# Autodesk Inventor assembly: suspensionsystem1
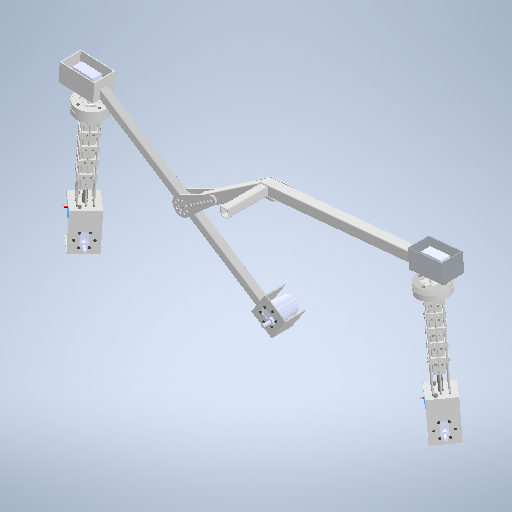
[picture p0: Inventor's stored thumbnail of the model, 512x512]
Saved by Autodesk Inventor 2025.2 (Build 292293000, 293)
## iProperties
Created: 2026-03-25
Part Number: suspensionsystem1
Document SubType Name: Assembly
Designer: hp
Author: hp
## Documents named in this file (31)
- C:\Users\hp\OneDrive\Desktop\Probitymechanicaldocs\suspensionsystem1.iam
- C:\Users\hp\OneDrive\Desktop\Probitymechanicaldocs\suspensionarms.ipt
- C:\Users\hp\OneDrive\Desktop\Probitymechanicaldocs\suspensionaxlebearing.ipt
- C:\Users\hp\OneDrive\Desktop\Probitymechanicaldocs\Controlarm.ipt
- C:\Users\hp\OneDrive\Desktop\Probitymechanicaldocs\rockershaft.ipt
- C:\Users\hp\OneDrive\Desktop\Probitymechanicaldocs\rockerwasher.ipt
- C:\Users\hp\OneDrive\Desktop\Probitymechanicaldocs\suspension2chassisarm.ipt
- C:\Users\hp\OneDrive\Desktop\Probitymechanicaldocs\150degreebracket.ipt
- C:\Users\hp\OneDrive\Desktop\Probitymechanicaldocs\rockerpivotarm.ipt
- C:\Users\hp\OneDrive\Desktop\Probitymechanicaldocs\finalturnmotorcasing.ipt
- C:\Users\hp\OneDrive\Desktop\Probitymechanicaldocs\finalturnmotorservo.ipt
- C:\Users\hp\OneDrive\Desktop\Probitymechanicaldocs\hexcoupling.ipt
- C:\Users\hp\OneDrive\Desktop\Probitymechanicaldocs\couplingload.ipt
- C:\Users\hp\OneDrive\Desktop\Probitymechanicaldocs\sleeve.ipt
- C:\Users\hp\OneDrive\Desktop\Probitymechanicaldocs\verticalaxle.ipt
- C:\Users\hp\OneDrive\Desktop\Probitymechanicaldocs\leadscrew.ipt
- C:\Users\hp\OneDrive\Desktop\Probitymechanicaldocs\leadscrewaxle.ipt
- C:\Users\hp\OneDrive\Desktop\Probitymechanicaldocs\RISE&Fallmotor.ipt
- C:\Users\hp\OneDrive\Desktop\Probitymechanicaldocs\spokes.ipt
- C:\Users\hp\OneDrive\Desktop\Probitymechanicaldocs\liftmotorfloor.ipt
- C:\Users\hp\OneDrive\Desktop\Probitymechanicaldocs\placeholderjoint.ipt
- C:\Users\hp\OneDrive\Desktop\Probitymechanicaldocs\impromptugraphitering.ipt
- C:\Users\hp\OneDrive\Desktop\Probitymechanicaldocs\Placeholderjointouterring.ipt
- C:\Users\hp\OneDrive\Desktop\Probitymechanicaldocs\drivemotorcasing.ipt
- C:\Users\hp\OneDrive\Desktop\Probitymechanicaldocs\extendeddrivemotorcasing.ipt
- C:\Users\hp\OneDrive\Desktop\Probitymechanicaldocs\finaldrivemotor.ipt
- C:\Users\hp\OneDrive\Desktop\Probitymechanicaldocs\150degreesidebracker.ipt
- C:\Users\hp\OneDrive\Desktop\Probitymechanicaldocs\suspension2chassis.ipt
- C:\Users\hp\OneDrive\Documents\Inventor\Content Center Files\R2025\en-US\ISO 4762(2)\ISO 4762 - M4 x 6ISO.ipt
- C:\Users\hp\OneDrive\Documents\Inventor\Content Center Files\R2025\en-US\ISO 7045  H\ISO 7045 - M2.5 x 3_ - 4.8 - H - ISO.ipt
- C:\Users\hp\OneDrive\Documents\Inventor\Content Center Files\R2025\en-US\ISO 1580\ISO 1580 - M2 x 2.5_.ipt
## Components (189 placed, 30 different names)
1. suspensionarms:1 — Rigid:8, Rotational:130, Rigid:32
2. suspensionaxlebearing:1 — Rotational:3
3. suspensionaxlebearing:2 — Cylindrical:1, Rotational:4, Rotational:130
4. Controlarm:1 — Rotational:9, Rotational:11, Rotational:131
5. Controlarm:2 — Cylindrical:11, Rotational:12, Rotational:132
6. rockershaft:1 — Cylindrical:1
7. rockerwasher:1 — Rotational:4, Rotational:6
8. rockerwasher:2 — Rotational:3, Rotational:5
9. suspensionaxlebearing:3 — Rotational:6, Rotational:11
10. suspensionaxlebearing:4 — Rotational:5, Cylindrical:11
11. suspension2chassisarm:1 — Rotational:9, Rotational:12, Rotational:72, Rotational:131, Rotational:132
12. 150degreebracket:1 — Rigid:16, Rotational:72, Rigid:24
13. rockerpivotarm:1 — Rigid:1, Rigid:16, Rigid:25
14. finalturnmotorcasing:1 — Rigid:1, Rigid:2
15. finalturnmotorservo:1 — Rigid:2, Rotational:13
16. hexcoupling:1 — Rotational:13, Rigid:3
17. couplingload:1 — Rigid:3, Rigid:4
18. sleeve:1 — Rotational:14, Rotational:15
19. verticalaxle:1 — Rigid:4, Rotational:14, Rotational:15, Rotational:16, Cylindrical:12, Rotational:17, Cylindrical:13, Rotational:18, Cylindrical:14, Rotational:19, Rigid:6, Rotational:29, Rotational:30, Rotational:31
20. leadscrew:1 — Rigid:6, Cylindrical:15
21. leadscrewaxle:1 — Rigid:5, Cylindrical:15
22. RISE&Fallmotor:1 — Rigid:5, Rotational:32, Rotational:33
23. sleeve:2 — Rotational:18, Cylindrical:14
24. sleeve:3 — Rotational:19, Rotational:29
25. sleeve:4 — Rotational:17, Cylindrical:13
26. sleeve:5 — Rotational:16, Cylindrical:12, Rigid:7
27. sleeve:6 — Rotational:30, Rotational:31
28. spokes:1 — Rotational:24
29. spokes:2 — Rotational:25
30. spokes:3 — Rotational:23
31. spokes:4 — Rotational:26
32. spokes:5 — Rotational:22
33. spokes:6 — Rotational:28
34. spokes:7 — Rotational:21
35. spokes:8 — Rotational:27
36. liftmotorfloor:1 — Rotational:21, Rotational:22, Rotational:23, Rotational:24, Rotational:25, Rotational:26, Rotational:27, Rotational:28, Rotational:32, Rotational:33, Rotational:62, Mate:5
37. placeholderjoint:1 — Rigid:7, Rotational:34
38. impromptugraphitering:1 — Rotational:34, Rotational:35, Rotational:102
39. Placeholderjointouterring:1 — Rotational:102
40. Placeholderjointouterring:2 — Rotational:35
41. drivemotorcasing:1 — Rigid:8, Rotational:63, Rotational:64, Insert:11, Insert:12, Insert:13, Insert:14, Insert:15, Insert:16
42. extendeddrivemotorcasing:1 — Rotational:62, Mate:5, Rotational:65, Rotational:66, Insert:17, Insert:18, Insert:19, Insert:20, Insert:21, Insert:22
43. finaldrivemotor:1 — Rotational:65, Rotational:66
44. finaldrivemotor:2 — Rotational:63, Rotational:64
45. 150degreesidebracker:1 — Rigid:24
46. suspension2chassis:1 — Rigid:25
47. finalturnmotorcasing:2 — Rigid:32
48. finalturnmotorservo:2
49. hexcoupling:2
50. couplingload:2
51. sleeve:7 — Insert:33, Insert:34, Insert:45, Insert:46
52. verticalaxle:2 — Insert:47, Insert:48
53. leadscrew:2
54. leadscrewaxle:2
55. RISE&Fallmotor:2
56. sleeve:8 — Insert:27, Insert:28, Insert:39, Insert:40
57. sleeve:9 — Insert:31, Insert:32, Insert:43, Insert:44
58. sleeve:10 — Insert:23, Insert:24, Insert:25, Insert:26, Insert:35, Insert:36, Insert:37, Insert:38
59. sleeve:11
60. sleeve:12 — Insert:29, Insert:30, Insert:41, Insert:42
61. spokes:9
62. spokes:10
63. spokes:11
64. spokes:12
65. spokes:13
66. spokes:14
67. spokes:15
68. spokes:16
69. liftmotorfloor:2
70. placeholderjoint:2
71. impromptugraphitering:2
72. Placeholderjointouterring:3
73. Placeholderjointouterring:4
74. extendeddrivemotorcasing:2 — Insert:5, Insert:6, Insert:7, Insert:8, Insert:9, Insert:10
75. finaldrivemotor:3
76. ISO 4762 M4 x 6:1
77. ISO 4762 M4 x 6:2
78. ISO 4762 M4 x 6:3
79. ISO 4762 M4 x 6:4
80. ISO 7045 H M2.5 x 3 - 4.8 - H:1 — Insert:5
81. ISO 7045 H M2.5 x 3 - 4.8 - H:2 — Insert:6
82. ISO 7045 H M2.5 x 3 - 4.8 - H:3 — Insert:7
83. ISO 7045 H M2.5 x 3 - 4.8 - H:4 — Insert:8
84. ISO 7045 H M2.5 x 3 - 4.8 - H:5 — Insert:9
85. ISO 7045 H M2.5 x 3 - 4.8 - H:6 — Insert:10
86. ISO 7045 H M2.5 x 3 - 4.8 - H:7 — Insert:11
87. ISO 7045 H M2.5 x 3 - 4.8 - H:8 — Insert:12
88. ISO 7045 H M2.5 x 3 - 4.8 - H:9 — Insert:13
89. ISO 7045 H M2.5 x 3 - 4.8 - H:10 — Insert:14
90. ISO 7045 H M2.5 x 3 - 4.8 - H:11 — Insert:15
91. ISO 7045 H M2.5 x 3 - 4.8 - H:12 — Insert:16
92. ISO 7045 H M2.5 x 3 - 4.8 - H:13 — Insert:17
93. ISO 7045 H M2.5 x 3 - 4.8 - H:14 — Insert:18
94. ISO 7045 H M2.5 x 3 - 4.8 - H:15 — Insert:19
95. ISO 7045 H M2.5 x 3 - 4.8 - H:16 — Insert:20
96. ISO 7045 H M2.5 x 3 - 4.8 - H:17 — Insert:21
97. ISO 7045 H M2.5 x 3 - 4.8 - H:18 — Insert:22
98. ISO 1580 M2 x 2.5:1
99. ISO 1580 M2 x 2.5:2
100. ISO 1580 M2 x 2.5:3
101. ISO 1580 M2 x 2.5:4
102. ISO 1580 M2 x 2.5:5
103. ISO 1580 M2 x 2.5:6
104. ISO 1580 M2 x 2.5:7
105. ISO 1580 M2 x 2.5:8
106. ISO 1580 M2 x 2.5:9
107. ISO 1580 M2 x 2.5:10
108. ISO 1580 M2 x 2.5:11
109. ISO 1580 M2 x 2.5:12
110. ISO 1580 M2 x 2.5:13
111. ISO 1580 M2 x 2.5:14
112. ISO 1580 M2 x 2.5:15
113. ISO 1580 M2 x 2.5:16
114. ISO 1580 M2 x 2.5:17
115. ISO 1580 M2 x 2.5:18
116. ISO 1580 M2 x 2.5:19
117. ISO 1580 M2 x 2.5:20
118. ISO 1580 M2 x 2.5:21
119. ISO 1580 M2 x 2.5:22
120. ISO 1580 M2 x 2.5:23
121. ISO 1580 M2 x 2.5:24
122. ISO 1580 M2 x 2.5:25
123. ISO 1580 M2 x 2.5:30
124. ISO 1580 M2 x 2.5:31
125. ISO 1580 M2 x 2.5:32
126. ISO 1580 M2 x 2.5:33
127. ISO 1580 M2 x 2.5:34
128. ISO 1580 M2 x 2.5:35
129. ISO 1580 M2 x 2.5:36
130. ISO 1580 M2 x 2.5:37
131. ISO 1580 M2 x 2.5:38
132. ISO 1580 M2 x 2.5:39
133. ISO 1580 M2 x 2.5:40
134. ISO 1580 M2 x 2.5:41
135. ISO 1580 M2 x 2.5:42
136. ISO 1580 M2 x 2.5:43
137. ISO 1580 M2 x 2.5:44
138. ISO 1580 M2 x 2.5:45
139. ISO 1580 M2 x 2.5:46
140. ISO 1580 M2 x 2.5:47
141. ISO 1580 M2 x 2.5:48
142. ISO 1580 M2 x 2.5:49
143. ISO 1580 M2 x 2.5:50
144. ISO 1580 M2 x 2.5:51
145. ISO 1580 M2 x 2.5:52
146. ISO 1580 M2 x 2.5:53
147. ISO 1580 M2 x 2.5:54
148. ISO 1580 M2 x 2.5:55
149. ISO 1580 M2 x 2.5:56
150. ISO 1580 M2 x 2.5:57
151. ISO 1580 M2 x 2.5:58
152. ISO 1580 M2 x 2.5:59
153. ISO 1580 M2 x 2.5:60
154. ISO 1580 M2 x 2.5:61
155. ISO 1580 M2 x 2.5:62
156. ISO 1580 M2 x 2.5:63
157. ISO 1580 M2 x 2.5:64 — Insert:23
158. ISO 1580 M2 x 2.5:65 — Insert:24
159. ISO 1580 M2 x 2.5:66 — Insert:25
160. ISO 1580 M2 x 2.5:67 — Insert:26
161. ISO 1580 M2 x 2.5:68 — Insert:27
162. ISO 1580 M2 x 2.5:69 — Insert:28
163. ISO 1580 M2 x 2.5:70 — Insert:29
164. ISO 1580 M2 x 2.5:71 — Insert:30
165. ISO 1580 M2 x 2.5:72 — Insert:31
166. ISO 1580 M2 x 2.5:73 — Insert:32
167. ISO 1580 M2 x 2.5:74 — Insert:33
168. ISO 1580 M2 x 2.5:75 — Insert:34
169. ISO 1580 M2 x 2.5:76 — Insert:35
170. ISO 1580 M2 x 2.5:77 — Insert:36
171. ISO 1580 M2 x 2.5:78 — Insert:37
172. ISO 1580 M2 x 2.5:79 — Insert:38
173. ISO 1580 M2 x 2.5:80 — Insert:39
174. ISO 1580 M2 x 2.5:81 — Insert:40
175. ISO 1580 M2 x 2.5:82 — Insert:41
176. ISO 1580 M2 x 2.5:83 — Insert:42
177. ISO 1580 M2 x 2.5:84 — Insert:43
178. ISO 1580 M2 x 2.5:85 — Insert:44
179. ISO 1580 M2 x 2.5:86 — Insert:45
180. ISO 1580 M2 x 2.5:87 — Insert:46
181. ISO 1580 M2 x 2.5:88 — Insert:47
182. ISO 1580 M2 x 2.5:26
183. ISO 1580 M2 x 2.5:27
184. ISO 1580 M2 x 2.5:28
185. ISO 1580 M2 x 2.5:29
186. ISO 1580 M2 x 2.5:89 — Insert:48
187. ISO 1580 M2 x 2.5:90
188. ISO 1580 M2 x 2.5:91
189. ISO 1580 M2 x 2.5:92
## Component patterns: (4 elements, first: ISO 1580 M2 x 2.5:26), (4 elements, first: ISO 1580 M2 x 2.5:89)
## Relationships (139: RevoluteJoint 65, Insert 44, WeldJoint 18, CylindricalJoint 10, Mate 2)
- Cylindrical:1: suspensionaxlebearing:2 ↔ rockershaft:1
- Rotational:3 [RevoluteJoint]: suspensionaxlebearing:1 ↔ rockerwasher:2
- Rotational:4 [RevoluteJoint]: suspensionaxlebearing:2 ↔ rockerwasher:1
- Rotational:5 [RevoluteJoint]: rockerwasher:2 ↔ suspensionaxlebearing:4
- Rotational:6 [RevoluteJoint]: rockerwasher:1 ↔ suspensionaxlebearing:3
- Rotational:9 [RevoluteJoint]: Controlarm:1 ↔ suspension2chassisarm:1
- Cylindrical:11: Controlarm:2 ↔ suspensionaxlebearing:4
- Rotational:11 [RevoluteJoint]: Controlarm:1 ↔ suspensionaxlebearing:3
- Rotational:12 [RevoluteJoint]: Controlarm:2 ↔ suspension2chassisarm:1
- Rigid:1 [WeldJoint]: rockerpivotarm:1 ↔ finalturnmotorcasing:1
- Rigid:2 [WeldJoint]: finalturnmotorcasing:1 ↔ finalturnmotorservo:1
- Rotational:13 [RevoluteJoint]: finalturnmotorservo:1 ↔ hexcoupling:1
- Rigid:3 [WeldJoint]: hexcoupling:1 ↔ couplingload:1
- Rigid:4 [WeldJoint]: couplingload:1 ↔ verticalaxle:1
- Rotational:14 [RevoluteJoint]: sleeve:1 ↔ verticalaxle:1
- Rotational:15 [RevoluteJoint]: sleeve:1 ↔ verticalaxle:1
- Rotational:16 [RevoluteJoint]: verticalaxle:1 ↔ sleeve:5
- Cylindrical:12: verticalaxle:1 ↔ sleeve:5
- Rotational:17 [RevoluteJoint]: verticalaxle:1 ↔ sleeve:4
- Cylindrical:13: verticalaxle:1 ↔ sleeve:4
- Rotational:18 [RevoluteJoint]: verticalaxle:1 ↔ sleeve:2
- Cylindrical:14: verticalaxle:1 ↔ sleeve:2
- Rotational:19 [RevoluteJoint]: verticalaxle:1 ↔ sleeve:3
- Rigid:5 [WeldJoint] (-4 mm): leadscrewaxle:1 ↔ RISE&Fallmotor:1
- Rigid:6 [WeldJoint]: verticalaxle:1 ↔ leadscrew:1
- Cylindrical:15: leadscrew:1 ↔ leadscrewaxle:1
- Rotational:21 [RevoluteJoint] (8 mm): spokes:7 ↔ liftmotorfloor:1
- Rotational:22 [RevoluteJoint] (8 mm): spokes:5 ↔ liftmotorfloor:1
- Rotational:23 [RevoluteJoint] (8 mm): spokes:3 ↔ liftmotorfloor:1
- Rotational:24 [RevoluteJoint] (8 mm): spokes:1 ↔ liftmotorfloor:1
- Rotational:25 [RevoluteJoint] (8 mm): spokes:2 ↔ liftmotorfloor:1
- Rotational:26 [RevoluteJoint] (8 mm): spokes:4 ↔ liftmotorfloor:1
- Rotational:27 [RevoluteJoint] (8 mm): spokes:8 ↔ liftmotorfloor:1
- Rotational:28 [RevoluteJoint] (8 mm): spokes:6 ↔ liftmotorfloor:1
- Rotational:29 [RevoluteJoint]: verticalaxle:1 ↔ sleeve:3
- Rotational:30 [RevoluteJoint]: verticalaxle:1 ↔ sleeve:6
- Rotational:31 [RevoluteJoint]: verticalaxle:1 ↔ sleeve:6
- Rotational:32 [RevoluteJoint]: RISE&Fallmotor:1 ↔ liftmotorfloor:1
- Rotational:33 [RevoluteJoint]: RISE&Fallmotor:1 ↔ liftmotorfloor:1
- Rigid:7 [WeldJoint]: sleeve:5 ↔ placeholderjoint:1
- Rotational:34 [RevoluteJoint]: placeholderjoint:1 ↔ impromptugraphitering:1
- Rotational:35 [RevoluteJoint]: impromptugraphitering:1 ↔ Placeholderjointouterring:2
- Rigid:8 [WeldJoint]: suspensionarms:1 ↔ drivemotorcasing:1
- Rotational:62 [RevoluteJoint]: liftmotorfloor:1 ↔ extendeddrivemotorcasing:1
- Mate:5: liftmotorfloor:1 ↔ extendeddrivemotorcasing:1
- Rotational:63 [RevoluteJoint]: drivemotorcasing:1 ↔ finaldrivemotor:2
- Rotational:64 [RevoluteJoint]: drivemotorcasing:1 ↔ finaldrivemotor:2
- Rotational:65 [RevoluteJoint]: extendeddrivemotorcasing:1 ↔ finaldrivemotor:1
- Rotational:66 [RevoluteJoint]: extendeddrivemotorcasing:1 ↔ finaldrivemotor:1
- Rigid:16 [WeldJoint]: 150degreebracket:1 ↔ rockerpivotarm:1
- Rotational:72 [RevoluteJoint]: suspension2chassisarm:1 ↔ 150degreebracket:1
- Rotational:102 [RevoluteJoint]: impromptugraphitering:1 ↔ Placeholderjointouterring:1
- Rotational:130 [RevoluteJoint]: suspensionarms:1 ↔ suspensionaxlebearing:2
- Rotational:131 [RevoluteJoint]: Controlarm:1 ↔ suspension2chassisarm:1
- Rotational:132 [RevoluteJoint]: Controlarm:2 ↔ suspension2chassisarm:1
- Rigid:24 [WeldJoint]: 150degreebracket:1 ↔ 150degreesidebracker:1
- Rigid:25 [WeldJoint]: rockerpivotarm:1 ↔ suspension2chassis:1
- [WeldJoint]: finalturnmotorcasing:2 ↔ finalturnmotorservo:2
- [RevoluteJoint]: finalturnmotorservo:2 ↔ hexcoupling:2
- [WeldJoint]: hexcoupling:2 ↔ couplingload:2
- [WeldJoint]: couplingload:2 ↔ verticalaxle:2
- [RevoluteJoint]: sleeve:7 ↔ verticalaxle:2
- [RevoluteJoint]: sleeve:7 ↔ verticalaxle:2
- [RevoluteJoint]: verticalaxle:2 ↔ sleeve:11
- [CylindricalJoint]: verticalaxle:2 ↔ sleeve:11
- [RevoluteJoint]: verticalaxle:2 ↔ sleeve:10
- [CylindricalJoint]: verticalaxle:2 ↔ sleeve:10
- [RevoluteJoint]: verticalaxle:2 ↔ sleeve:8
- [CylindricalJoint]: verticalaxle:2 ↔ sleeve:8
- [RevoluteJoint]: verticalaxle:2 ↔ sleeve:9
- [WeldJoint] (-4 mm): leadscrewaxle:2 ↔ RISE&Fallmotor:2
- [WeldJoint]: verticalaxle:2 ↔ leadscrew:2
- [CylindricalJoint]: leadscrew:2 ↔ leadscrewaxle:2
- [RevoluteJoint] (8 mm): spokes:15 ↔ liftmotorfloor:2
- [RevoluteJoint] (8 mm): spokes:13 ↔ liftmotorfloor:2
- [RevoluteJoint] (8 mm): spokes:11 ↔ liftmotorfloor:2
- [RevoluteJoint] (8 mm): spokes:9 ↔ liftmotorfloor:2
- [RevoluteJoint] (8 mm): spokes:10 ↔ liftmotorfloor:2
- [RevoluteJoint] (8 mm): spokes:12 ↔ liftmotorfloor:2
- [RevoluteJoint] (8 mm): spokes:16 ↔ liftmotorfloor:2
- [RevoluteJoint] (8 mm): spokes:14 ↔ liftmotorfloor:2
- [RevoluteJoint]: verticalaxle:2 ↔ sleeve:9
- [RevoluteJoint]: verticalaxle:2 ↔ sleeve:12
- [RevoluteJoint]: verticalaxle:2 ↔ sleeve:12
- [RevoluteJoint]: RISE&Fallmotor:2 ↔ liftmotorfloor:2
- [RevoluteJoint]: RISE&Fallmotor:2 ↔ liftmotorfloor:2
- [WeldJoint]: sleeve:11 ↔ placeholderjoint:2
- [RevoluteJoint]: placeholderjoint:2 ↔ impromptugraphitering:2
- [RevoluteJoint]: impromptugraphitering:2 ↔ Placeholderjointouterring:4
- [RevoluteJoint]: liftmotorfloor:2 ↔ extendeddrivemotorcasing:2
- [Mate]: liftmotorfloor:2 ↔ extendeddrivemotorcasing:2
- [RevoluteJoint]: extendeddrivemotorcasing:2 ↔ finaldrivemotor:3
- [RevoluteJoint]: extendeddrivemotorcasing:2 ↔ finaldrivemotor:3
- [RevoluteJoint]: impromptugraphitering:2 ↔ Placeholderjointouterring:3
- Rigid:32 [WeldJoint]: suspensionarms:1 ↔ finalturnmotorcasing:2
- Insert:5: extendeddrivemotorcasing:2 ↔ ISO 7045 H M2.5 x 3 - 4.8 - H:1
- Insert:6: extendeddrivemotorcasing:2 ↔ ISO 7045 H M2.5 x 3 - 4.8 - H:2
- Insert:7: extendeddrivemotorcasing:2 ↔ ISO 7045 H M2.5 x 3 - 4.8 - H:3
- Insert:8: extendeddrivemotorcasing:2 ↔ ISO 7045 H M2.5 x 3 - 4.8 - H:4
- Insert:9: extendeddrivemotorcasing:2 ↔ ISO 7045 H M2.5 x 3 - 4.8 - H:5
- Insert:10: extendeddrivemotorcasing:2 ↔ ISO 7045 H M2.5 x 3 - 4.8 - H:6
- Insert:11: drivemotorcasing:1 ↔ ISO 7045 H M2.5 x 3 - 4.8 - H:7
- Insert:12: drivemotorcasing:1 ↔ ISO 7045 H M2.5 x 3 - 4.8 - H:8
- Insert:13: drivemotorcasing:1 ↔ ISO 7045 H M2.5 x 3 - 4.8 - H:9
- Insert:14: drivemotorcasing:1 ↔ ISO 7045 H M2.5 x 3 - 4.8 - H:10
- Insert:15: drivemotorcasing:1 ↔ ISO 7045 H M2.5 x 3 - 4.8 - H:11
- Insert:16: drivemotorcasing:1 ↔ ISO 7045 H M2.5 x 3 - 4.8 - H:12
- Insert:17: extendeddrivemotorcasing:1 ↔ ISO 7045 H M2.5 x 3 - 4.8 - H:13
- Insert:18: extendeddrivemotorcasing:1 ↔ ISO 7045 H M2.5 x 3 - 4.8 - H:14
- Insert:19: extendeddrivemotorcasing:1 ↔ ISO 7045 H M2.5 x 3 - 4.8 - H:15
- Insert:20: extendeddrivemotorcasing:1 ↔ ISO 7045 H M2.5 x 3 - 4.8 - H:16
- Insert:21: extendeddrivemotorcasing:1 ↔ ISO 7045 H M2.5 x 3 - 4.8 - H:17
- Insert:22: extendeddrivemotorcasing:1 ↔ ISO 7045 H M2.5 x 3 - 4.8 - H:18
- Insert:23: sleeve:10 ↔ ISO 1580 M2 x 2.5:64
- Insert:24: sleeve:10 ↔ ISO 1580 M2 x 2.5:65
- Insert:25: sleeve:10 ↔ ISO 1580 M2 x 2.5:66
- Insert:26: sleeve:10 ↔ ISO 1580 M2 x 2.5:67
- Insert:27: sleeve:8 ↔ ISO 1580 M2 x 2.5:68
- Insert:28: sleeve:8 ↔ ISO 1580 M2 x 2.5:69
- Insert:29: sleeve:12 ↔ ISO 1580 M2 x 2.5:70
- Insert:30: sleeve:12 ↔ ISO 1580 M2 x 2.5:71
- Insert:31: sleeve:9 ↔ ISO 1580 M2 x 2.5:72
- Insert:32: sleeve:9 ↔ ISO 1580 M2 x 2.5:73
- Insert:33: sleeve:7 ↔ ISO 1580 M2 x 2.5:74
- Insert:34: sleeve:7 ↔ ISO 1580 M2 x 2.5:75
- Insert:35: sleeve:10 ↔ ISO 1580 M2 x 2.5:76
- Insert:36: sleeve:10 ↔ ISO 1580 M2 x 2.5:77
- Insert:37: sleeve:10 ↔ ISO 1580 M2 x 2.5:78
- Insert:38: sleeve:10 ↔ ISO 1580 M2 x 2.5:79
- Insert:39: sleeve:8 ↔ ISO 1580 M2 x 2.5:80
- Insert:40: sleeve:8 ↔ ISO 1580 M2 x 2.5:81
- Insert:41: sleeve:12 ↔ ISO 1580 M2 x 2.5:82
- Insert:42: sleeve:12 ↔ ISO 1580 M2 x 2.5:83
- Insert:43: sleeve:9 ↔ ISO 1580 M2 x 2.5:84
- Insert:44: sleeve:9 ↔ ISO 1580 M2 x 2.5:85
- Insert:45: sleeve:7 ↔ ISO 1580 M2 x 2.5:86
- Insert:46: sleeve:7 ↔ ISO 1580 M2 x 2.5:87
- Insert:47: verticalaxle:2 ↔ ISO 1580 M2 x 2.5:88
- Insert:48: verticalaxle:2 ↔ ISO 1580 M2 x 2.5:89
## Named parameters: d392_d186 = 0 mm, d393_d187 = 90 deg, d394_d188 = 0 mm, d395_d195 = 0 mm, d396_d196 = 90 deg, d397_d197 = 0 mm, d398_d198 = 180 deg, d399_d105 = 0 mm, d400_d106 = 0 mm, d401_d107 = 16.418665 deg, d402_d108 = 0 mm, d403_d109 = 35.17501 deg, d404_d79 = 8 mm, d405_d80 = 177.875479 deg, d406_d81 = 8 mm, d407_d82 = -132.013809 deg, d408_d83 = 8 mm, d409_d84 = 124.362439 deg, d410_d85 = 8 mm, d411_d86 = 166.937725 deg, d412_d87 = 8 mm, d413_d88 = 134.09897 deg, d414_d89 = 8 mm, d415_d90 = -51.929464 deg, d416_d91 = 8 mm, d417_d92 = 115.673908 deg, d418_d93 = 0 mm, d419_d94 = -90 deg, d420_d95 = 0 mm, d421_d96 = 180 deg, d422_d97 = 0 mm, d423_d98 = 90 deg, d424_d100 = 0 mm, d425_d101 = 180 deg, d426_d102 = 0 mm, d427_d103 = -112.112234 deg, d428_d57 = 180 deg, d429_d58 = 2.5 mm, d430_d59 = 0 mm, d431_d60 = 90 deg, d432_d61 = -90 deg, d433_d62 = -5 mm, d434_d63 = 0 mm, d435_d64 = 90 deg, d436_d65 = 90 deg, d437_d66 = -5 mm, d438_d67 = 0 mm, d439_d68 = 0 deg, d440_d73 = -4 mm, d441_d74 = 0 mm, d442_d75 = -88.338929 deg, d443_d76 = 30.54603 mm, d444_d77 = 8 mm, d445_d78 = 159.367241 deg, d446_d46 = 0 mm, d447_d47 = 0 mm, d448_d48 = 170.413895 deg, d449_d49 = 0 mm, d450_d50 = 0 mm, d451_d51 = 0 mm, d452_d52 = 0 deg, d453_d53 = 0 mm, d454_d54 = 0 deg, d455_d55 = 0 mm, d456_d56 = 90 deg, d457_d307 = 0 mm, d458_d308 = 91.23069 deg
